# Autodesk Inventor assembly: OfflineExtruderRight
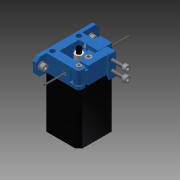
[picture p0: Inventor's stored thumbnail of the model, 180x180]
Saved by Autodesk Inventor 2015 SP1 (Build 190203100, 203)
## iProperties
Created: 2015-04-29
Part Number: OfflineExtruderRight
Document SubType Name: Assembly
Designer: Jack
Author: Jack
## Documents named in this file (14)
- C:\Users\Jack\ownCloud\Projects\CrossBot\InventorModel\Extruder\OfflineBowdenExtruder\OfflineExtruderRight.iam
- C:\Users\Jack\ownCloud\Projects\CrossBot\InventorModel\Extruder\OfflineBowdenExtruder\OfflineBowdenExtruder.ipt
- C:\Users\Jack\ownCloud\Projects\CrossBot\InventorModel\Electronics\Motors\StepperMotorNema17x60mm.ipt
- C:\Users\Jack\ownCloud\Projects\CrossBot\InventorModel\Hardware\Extruder\DriveGearMK8.ipt
- C:\Users\Jack\ownCloud\Projects\CrossBot\InventorModel\Extruder\OfflineBowdenExtruder\OfflineBowdenExtruderIdler.ipt
- C:\Users\Jack\ownCloud\Projects\CrossBot\InventorModel\Hardware\Bearing\BearingRadialBall\BearingRadialBall624zz.ipt
- C:\Users\Jack\ownCloud\Projects\CrossBot\InventorModel\Hardware\BoltWashers\BoltWasher4\BoltWasher4x10.iam
- C:\Users\Jack\ownCloud\Projects\CrossBot\InventorModel\Hardware\Bolts\SHCS\SHCS3\SHCS3x12.ipt
- C:\Users\Jack\ownCloud\Projects\CrossBot\InventorModel\Hardware\Bolts\SHCS\SHCS3\SHCS3x20.ipt
- C:\Users\Jack\ownCloud\Projects\CrossBot\InventorModel\Hardware\Bolts\SHCS\SHCS4\SHCS4x12.ipt
- C:\Users\Jack\ownCloud\Projects\CrossBot\InventorModel\Hardware\Nuts\Nut4.ipt
- C:\Users\Jack\ownCloud\Projects\CrossBot\InventorModel\Extruder\OfflineBowdenExtruder\OfflineBowdenExtruderSpringHandle.ipt
- C:\Users\Jack\ownCloud\Projects\CrossBot\InventorModel\Hardware\Bolts\SHCS\SHCS4\SHCS4x45.ipt
- C:\Users\Jack\ownCloud\Projects\CrossBot\STLs\Extruder\FilamentStrip.ipt
## Components (18 placed, 13 different names)
1. OfflineBowdenExtruder:1 — Mate:1, Mate:2, Mate:3, Mate:4, Mate:7, Mate:8, Mate:11, Mate:12, Mate:13, Mate:14, Mate:15, Mate:16, Mate:17, Mate:18, Mate:19, Mate:20, Mate:25, Mate:26, Angle:2, Mate:27, Mate:28, Angle:3, Mate:29, Mate:30, Mate:31, Mate:32, Mate:34
2. StepperMotorNema17x60mm:1 — Mate:1, Mate:2, Mate:3, Mate:4, Mate:5, Mate:6
3. DriveGearMK8:1 — Mate:5, Mate:6
4. OfflineBowdenExtruderIdler:1 — Mate:7, Mate:8, Mate:9, Mate:10, Mate:21, Mate:22, Angle:1, Mate:24
5. BearingRadialBall624zz:1 — Mate:9, Mate:10
6. BoltWasher4x10:1 [sub-assembly] — Mate:11, Mate:14
7. BoltWasher4x10:2 [sub-assembly] — Mate:12, Mate:13
8. SHCS3x12:1 — Mate:15, Mate:17
9. SHCS3x12:2 — Mate:16, Mate:18
10. SHCS3x20:1 — Mate:19, Mate:20
11. SHCS4x12:1 — Mate:21, Mate:22, Mate:23
12. Nut4:1 — Mate:23, Angle:1, Mate:24
13. Nut4:2 — Mate:25, Mate:26, Angle:2
14. Nut4:3 — Mate:27, Mate:28, Angle:3
15. OfflineBowdenExtruderSpringHandle:1 — Mate:29, Mate:30, Mate:33
16. SHCS4x45:1 — Mate:31, Flush:1
17. SHCS4x45:2 — Mate:32, Mate:33, Flush:1
18. FilamentStrip:1 — Mate:34
## Relationships (38: Mate 34, Angle 3, Flush 1)
- Mate:1: OfflineBowdenExtruder:1 ↔ StepperMotorNema17x60mm:1
- Mate:2: OfflineBowdenExtruder:1 ↔ StepperMotorNema17x60mm:1
- Mate:3: OfflineBowdenExtruder:1 ↔ StepperMotorNema17x60mm:1
- Mate:4: OfflineBowdenExtruder:1 ↔ StepperMotorNema17x60mm:1
- Mate:5: StepperMotorNema17x60mm:1 ↔ DriveGearMK8:1
- Mate:6 (5 mm): StepperMotorNema17x60mm:1 ↔ DriveGearMK8:1
- Mate:7: OfflineBowdenExtruder:1 ↔ OfflineBowdenExtruderIdler:1
- Mate:8 (0.2 mm): OfflineBowdenExtruder:1 ↔ OfflineBowdenExtruderIdler:1
- Mate:9: OfflineBowdenExtruderIdler:1 ↔ BearingRadialBall624zz:1
- Mate:10: OfflineBowdenExtruderIdler:1 ↔ BearingRadialBall624zz:1
- Mate:11: OfflineBowdenExtruder:1 ↔ BoltWasher4x10:1
- Mate:12: OfflineBowdenExtruder:1 ↔ BoltWasher4x10:2
- Mate:13: OfflineBowdenExtruder:1 ↔ BoltWasher4x10:2
- Mate:14: OfflineBowdenExtruder:1 ↔ BoltWasher4x10:1
- Mate:15: OfflineBowdenExtruder:1 ↔ SHCS3x12:1
- Mate:16: OfflineBowdenExtruder:1 ↔ SHCS3x12:2
- Mate:17: OfflineBowdenExtruder:1 ↔ SHCS3x12:1
- Mate:18: OfflineBowdenExtruder:1 ↔ SHCS3x12:2
- Mate:19: OfflineBowdenExtruder:1 ↔ SHCS3x20:1
- Mate:20: OfflineBowdenExtruder:1 ↔ SHCS3x20:1
- Mate:21: OfflineBowdenExtruderIdler:1 ↔ SHCS4x12:1
- Mate:22: OfflineBowdenExtruderIdler:1 ↔ SHCS4x12:1
- Mate:23: SHCS4x12:1 ↔ Nut4:1
- Angle:1 (0 deg): OfflineBowdenExtruderIdler:1 ↔ Nut4:1
- Mate:24: OfflineBowdenExtruderIdler:1 ↔ Nut4:1
- Mate:25: OfflineBowdenExtruder:1 ↔ Nut4:2
- Mate:26: OfflineBowdenExtruder:1 ↔ Nut4:2
- Angle:2 (0 deg): OfflineBowdenExtruder:1 ↔ Nut4:2
- Mate:27: OfflineBowdenExtruder:1 ↔ Nut4:3
- Mate:28: OfflineBowdenExtruder:1 ↔ Nut4:3
- Angle:3 (0 deg): OfflineBowdenExtruder:1 ↔ Nut4:3
- Mate:29: OfflineBowdenExtruder:1 ↔ OfflineBowdenExtruderSpringHandle:1
- Mate:30: OfflineBowdenExtruder:1 ↔ OfflineBowdenExtruderSpringHandle:1
- Mate:31: OfflineBowdenExtruder:1 ↔ SHCS4x45:1
- Mate:32: OfflineBowdenExtruder:1 ↔ SHCS4x45:2
- Mate:33 (14 mm): OfflineBowdenExtruderSpringHandle:1 ↔ SHCS4x45:2
- Flush:1: SHCS4x45:1 ↔ SHCS4x45:2
- Mate:34: OfflineBowdenExtruder:1 ↔ FilamentStrip:1
